# Autodesk Inventor assembly: Rubiks Arm Assembly
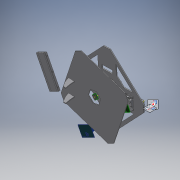
[picture p0: Inventor's stored thumbnail of the model, 180x180]
Saved by Autodesk Inventor 2017 (Build 210142000, 142)
## iProperties
Created: 2018-11-23
Part Number: Rubiks Arm Assembly
Document SubType Name: Assembly
Designer: Eric the Great
Author: Eric the Great
## Documents named in this file (21)
- C:\Users\Eric the Great\Documents\Cornell University\ECE 5725\Final Project\Rubiks Arm Assembly.iam
- C:\Users\Eric the Great\Documents\Cornell University\Kirstin Research\axle.ipt
- C:\Users\Eric the Great\Documents\Cornell University\ECE 5725\Final Project\Nema 17.ipt
- C:\Users\Eric the Great\Documents\Cornell University\ECE 5725\Final Project\Solenoid.ipt
- C:\Users\Eric the Great\Documents\Cornell University\ECE 5725\Final Project\8mmx22mm bearing.ipt
- C:\Users\Eric the Great\Documents\Cornell University\ECE 5725\Final Project\Claw.ipt
- C:\Users\Eric the Great\Documents\Cornell University\ECE 5725\Final Project\Base Plate.ipt
- C:\Users\Eric the Great\Documents\Cornell University\ECE 5725\Final Project\piston.ipt
- C:\Users\Eric the Great\Documents\Cornell University\ECE 5725\Final Project\solenoid base.ipt
- C:\Users\Eric the Great\Documents\Cornell University\ECE 5725\Final Project\solenoid piston.ipt
- C:\Users\Eric the Great\Documents\Cornell University\ECE 5725\Final Project\bearing block.ipt
- C:\Users\Eric the Great\Documents\Cornell University\ECE 5725\Final Project\stepper mount.ipt
- C:\Users\Eric the Great\Documents\Cornell University\ECE 5725\Final Project\Rubiks Arm Assembly\Design Accelerator\Spur Gear22.ipt
- C:\Users\Eric the Great\Documents\Cornell University\ECE 5725\Final Project\Rubiks Arm Assembly\Design Accelerator\Spur Gear12.ipt
- C:\Users\Eric the Great\Documents\Cornell University\ECE 5725\Final Project\bottom plate.ipt
- C:\Users\Eric the Great\Documents\Cornell University\ECE 5725\Final Project\Rpi3Bplus.ipt
- C:\Users\Eric the Great\Documents\Cornell University\ECE 5725\Final Project\RspCameraMia.ipt
- C:\Users\Eric the Great\Documents\Cornell University\ECE 5725\Final Project\leg.ipt
- C:\Users\Eric the Great\Documents\Cornell University\ECE 5725\Final Project\relay.ipt
- C:\Users\Eric the Great\Documents\Cornell University\ECE 5725\Final Project\BREADBOARD 60 ROW.ipt
- C:\Users\Eric the Great\Documents\Cornell University\ECE 5725\Final Project\Rubik's Cube.ipt
## Components (23 placed, 20 different names)
1. Rubik's Cube:1 — Mate:77, Mate:78, Mate:79, Mate:80
2. Base Plate:1 — Mate:51, Mate:52, Mate:60, Flush:4, Flush:5, Flush:6, Flush:7, Mate:67, Mate:73, Flush:79, Flush:80, Flush:81, Flush:82, Flush:83, Flush:84
3. piston:1
4. solenoid base:1
5. bottom plate:1 — Mate:67, Mate:68, Mate:70, Mate:71, Flush:8, Flush:11, Mate:75, Mate:76, Flush:78
6. Rpi3Bplus:1 — Mate:68, Flush:8
7. RspCameraMia:1 — Mate:69, Mate:71
8. Nema 17:1 — Mate:31, Mate:42, Mate:54, Mate:55, Mate:59, Mate:82
9. stepper mount:1 — Mate:59, Mate:60, Flush:84, Mate:82
10. Spur Gear2:1 — Mate:54, Mate:55
11. Solenoid:1 — Mate:42, Mate:62
12. solenoid piston:1 — Mate:61, Mate:63
13. 8mmx22mm bearing:2 — Mate:2, Mate:48
14. bearing block:2 — Mate:48, Mate:52, Mate:53
15. Spur Gear1:1 — Mate:56, Mate:57
16. 8mmx22mm bearing:1 — Mate:1, Mate:50
17. axle:1 — Mate:1, Mate:2, Mate:18, Mate:27, Mate:56, Mate:57, Mate:61, Mate:62, Mate:63, Mate:77, Mate:81
18. bearing block:3 — Mate:50, Mate:51, Mate:53, Mate:81, Flush:83
19. Claw:1 — Mate:18, Mate:27
20. leg:1 — Mate:72, Flush:9, Flush:10, Symmetry:3
21. leg:2 — Mate:72, Flush:9, Flush:10, Mate:73, Symmetry:3
22. relay:1 — Flush:11, Mate:75
23. BREADBOARD 60 ROW:1 — Mate:76, Flush:78
## Relationships (55: Mate 35, Flush 15, Symmetry 5)
- Mate:1: 8mmx22mm bearing:1 ↔ axle:1
- Mate:2: 8mmx22mm bearing:2 ↔ axle:1
- Mate:18: axle:1 ↔ Claw:1
- Mate:27: axle:1 ↔ Claw:1
- Mate:31: Nema 17:1
- Mate:42: Nema 17:1 ↔ Solenoid:1
- Mate:48: 8mmx22mm bearing:2 ↔ bearing block:2
- Mate:50: 8mmx22mm bearing:1 ↔ bearing block:3
- Mate:51: Base Plate:1 ↔ bearing block:3
- Mate:52: Base Plate:1 ↔ bearing block:2
- Mate:53 (39 mm): bearing block:2 ↔ bearing block:3
- Mate:54 (3 mm): Nema 17:1 ↔ Spur Gear2:1
- Mate:55: Nema 17:1 ↔ Spur Gear2:1
- Mate:56: Spur Gear1:1 ↔ axle:1
- Mate:57: Spur Gear1:1 ↔ axle:1
- Mate:59: Nema 17:1 ↔ stepper mount:1
- Mate:60: Base Plate:1 ↔ stepper mount:1
- Mate:61: solenoid piston:1 ↔ axle:1
- Mate:62: Solenoid:1 ↔ axle:1
- Mate:63: solenoid piston:1 ↔ axle:1
- Flush:4: Base Plate:1
- Flush:5: Base Plate:1
- Symmetry:1
- Flush:6: Base Plate:1
- Flush:7: Base Plate:1
- Symmetry:2
- Mate:67 (69.85 mm): Base Plate:1 ↔ bottom plate:1
- Mate:68 (5 mm): bottom plate:1 ↔ Rpi3Bplus:1
- Mate:69: RspCameraMia:1
- Mate:70: bottom plate:1
- Mate:71: bottom plate:1 ↔ RspCameraMia:1
- Flush:8 (20 mm): bottom plate:1 ↔ Rpi3Bplus:1
- Mate:72 (70 mm): leg:1 ↔ leg:2
- Flush:9: leg:1 ↔ leg:2
- Flush:10: leg:1 ↔ leg:2
- Mate:73: Base Plate:1 ↔ leg:2
- Symmetry:3: leg:1 ↔ leg:2
- Flush:11 (30 mm): bottom plate:1 ↔ relay:1
- Mate:75: bottom plate:1 ↔ relay:1
- Mate:76: bottom plate:1 ↔ BREADBOARD 60 ROW:1
- Flush:78 (10 mm): bottom plate:1 ↔ BREADBOARD 60 ROW:1
- Mate:77: Rubik's Cube:1 ↔ axle:1
- Mate:78: Rubik's Cube:1
- Flush:79: Base Plate:1
- Flush:80: Base Plate:1
- Symmetry:4
- Mate:79: Rubik's Cube:1
- Flush:81: Base Plate:1
- Flush:82: Base Plate:1
- Symmetry:5
- Mate:80: Rubik's Cube:1
- Mate:81: axle:1 ↔ bearing block:3
- Flush:83 (1 mm): Base Plate:1 ↔ bearing block:3
- Flush:84: Base Plate:1 ↔ stepper mount:1
- Mate:82: Nema 17:1 ↔ stepper mount:1
